# Autodesk Inventor assembly: NotchClickerAsm
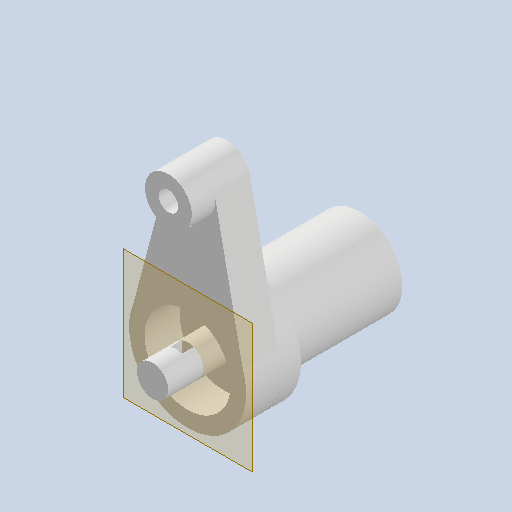
[picture p0: Inventor's stored thumbnail of the model, 512x512]
Saved by Autodesk Inventor 2022 (Build 260153000, 153)
## iProperties
Created: 2021-07-10
Part Number: NotchClickerAsm
Document SubType Name: Assembly
Designer: teh18
Author: teh18
## Documents named in this file (3)
- C:\Users\teh18\OneDrive\BVE Controller\r68-bve-mascon\NotchClickerAsm.iam
- C:\Users\teh18\OneDrive\BVE Controller\r68-bve-mascon\NotchClicker\ClickHolder.ipt
- C:\Users\teh18\OneDrive\BVE Controller\r68-bve-mascon\NotchClicker\ClickSpringBacking.ipt
## Components (2 placed, 2 different names)
1. ClickHolder:1 — Flush:1, Mate:1
2. ClickSpringBacking:1 — Flush:1, Mate:1
## Relationships (2: Flush 1, Mate 1)
- Flush:1: ClickHolder:1 ↔ ClickSpringBacking:1
- Mate:1: ClickHolder:1 ↔ ClickSpringBacking:1
